# Autodesk Inventor assembly: Middle_Gear
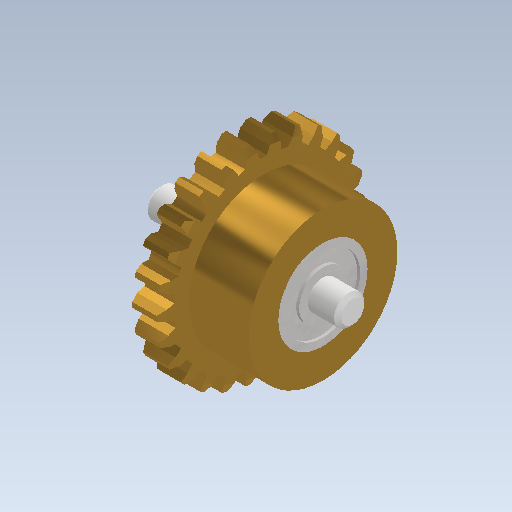
[picture p0: Inventor's stored thumbnail of the model, 512x512]
Saved by Autodesk Inventor 2020.4 (Build 244396000, 396)
## iProperties
Created: 2021-02-25
Part Number: Middle_Gear
Document SubType Name: Assembly
Designer: Acer
Author: Acer
## Documents named in this file (4)
- G:\Meu Drive\RobôCIn\Mecânica\SSL\2021\Inventor\first_floor\dribbler-3-gears\Middle_Gear.iam
- G:\Meu Drive\RobôCIn\Mecânica\SSL\2021\Inventor\first_floor\dribbler-3-gears\Ritzel schmal z26_machined.ipt
- G:\Meu Drive\RobôCIn\Mecânica\SSL\2021\Inventor\first_floor\dribbler-3-gears\Kugellager 692-ZZ.ipt
- G:\Meu Drive\RobôCIn\Mecânica\SSL\2021\Inventor\first_floor\dribbler-3-gears\pino.ipt
## Components (4 placed, 3 different names)
1. Ritzel schmal z=26:1 — Mate:1, Mate:2, Flush:1, Flush:2
2. Kugellager 692-ZZ:1 — Mate:1, Mate:3, Mate:4
3. Kugellager 692-ZZ:2 — Mate:2, Flush:1, Mate:3
4. pino:1 — Mate:4, Flush:2
## Relationships (6: Mate 4, Flush 2)
- Mate:1: Ritzel schmal z=26:1 ↔ Kugellager 692-ZZ:1
- Mate:2: Ritzel schmal z=26:1 ↔ Kugellager 692-ZZ:2
- Flush:1: Ritzel schmal z=26:1 ↔ Kugellager 692-ZZ:2
- Mate:3: Kugellager 692-ZZ:1 ↔ Kugellager 692-ZZ:2
- Mate:4: Kugellager 692-ZZ:1 ↔ pino:1
- Flush:2 (-2 mm): Ritzel schmal z=26:1 ↔ pino:1
